# Autodesk Inventor assembly: Chassisv1
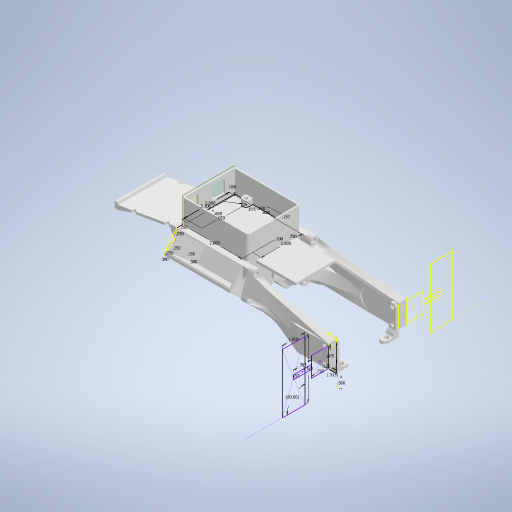
[picture p0: Inventor's stored thumbnail of the model, 512x512]
Saved by Autodesk Inventor 2024 (Build 280153020, 153B)
## iProperties
Created: 2024-03-25
Part Number: Chassisv1
Document SubType Name: Assembly
Designer: lvrectanus0
Author: lvrectanus0
## Documents named in this file (8)
- C:\Users\lvrectanus0\Documents\Github\SPARKLabs-ArduinoProjects\project\CAD\Autodesk\Chassisv1.iam
- C:\Users\lvrectanus0\Documents\Github\SPARKLabs-ArduinoProjects\project\CAD\Autodesk\ArduinoHolder-v2.ipt
- C:\Users\lvrectanus0\Documents\Github\SPARKLabs-ArduinoProjects\project\CAD\Autodesk\BatteryMount-v1.ipt
- C:\Users\lvrectanus0\Documents\Github\SPARKLabs-ArduinoProjects\project\CAD\Autodesk\BreadboardHolderv1.ipt
- C:\Users\lvrectanus0\Documents\Github\SPARKLabs-ArduinoProjects\project\CAD\Autodesk\MotorController-v1.ipt
- C:\Users\lvrectanus0\Documents\Github\SPARKLabs-ArduinoProjects\project\CAD\Autodesk\Sensor Mount.ipt
- C:\Users\lvrectanus0\Documents\Github\SPARKLabs-ArduinoProjects\project\CAD\Autodesk\MotorController-v1_MIR.ipt
- C:\Users\lvrectanus0\Documents\Github\SPARKLabs-ArduinoProjects\project\CAD\Autodesk\Exports\MotorControllerHolder-v1.ipt
## Components (8 placed, 7 different names)
1. ArduinoHolder-v2:1 — Flush:1, Flush:2
2. BatteryMount-v1:1 — Flush:1, Flush:2, Flush:3, Flush:4, Mate:1, Mate:2, Mate:3, Flush:7, Flush:8
3. BreadboardHolderv1:1 — Flush:3
4. MotorController-v1:1 — Flush:4, Flush:5, Flush:6
5. Sensor Mount:1 — Flush:5, Flush:6
6. MotorController-v1_MIR:1 — Mate:1, Mate:2, Mate:3, Mate:4, Mate:5, Mate:6
7. Sensor Mount:2 — Mate:4, Mate:5, Mate:6
8. MotorControllerHolder-v1:1 — Flush:7, Flush:8
## Relationships (14: Flush 8, Mate 6)
- Flush:1: ArduinoHolder-v2:1 ↔ BatteryMount-v1:1
- Flush:2: ArduinoHolder-v2:1 ↔ BatteryMount-v1:1
- Flush:3: BatteryMount-v1:1 ↔ BreadboardHolderv1:1
- Flush:4: BatteryMount-v1:1 ↔ MotorController-v1:1
- Flush:5: MotorController-v1:1 ↔ Sensor Mount:1
- Flush:6: MotorController-v1:1 ↔ Sensor Mount:1
- Mate:1: BatteryMount-v1:1 ↔ MotorController-v1_MIR:1
- Mate:2: BatteryMount-v1:1 ↔ MotorController-v1_MIR:1
- Mate:3: BatteryMount-v1:1 ↔ MotorController-v1_MIR:1
- Mate:4: MotorController-v1_MIR:1 ↔ Sensor Mount:2
- Mate:5: MotorController-v1_MIR:1 ↔ Sensor Mount:2
- Mate:6: MotorController-v1_MIR:1 ↔ Sensor Mount:2
- Flush:7: BatteryMount-v1:1 ↔ MotorControllerHolder-v1:1
- Flush:8: BatteryMount-v1:1 ↔ MotorControllerHolder-v1:1
